# Autodesk Inventor assembly: CaseAssembly
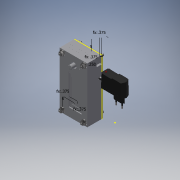
[picture p0: Inventor's stored thumbnail of the model, 180x180]
Saved by Autodesk Inventor 2018 (Build 220112000, 112)
## iProperties
Created: 2020-03-31
Part Number: CaseAssembly
Document SubType Name: Assembly
Designer: emile
Author: emile
## Documents named in this file (11)
- C:\Users\emile\OneDrive\Documents\GitHub\VentilatorCovid19\Respirator\MultiLine\ArduinoCase\CaseAssembly.iam
- C:\Users\emile\OneDrive\Documents\Inventor\Respirator\MultiLine\AC 12V 1A ADAPTER.ipt
- C:\Users\emile\OneDrive\Documents\Inventor\Respirator\MultiLine\ArduinoMega_STEP_AP203.ipt
- C:\Users\emile\OneDrive\Documents\Inventor\Respirator\MultiLine\Ramps 1.4 2004 LCD PRUSA RepRap.ipt
- C:\Users\emile\OneDrive\Documents\Inventor\Respirator\MultiLine\RelayBoard.ipt
- C:\Users\emile\OneDrive\Documents\GitHub\VentilatorCovid19\Respirator\MultiLine\ArduinoCase\FrontPanel.ipt
- C:\Users\emile\OneDrive\Documents\GitHub\VentilatorCovid19\Respirator\MultiLine\ArduinoCase\CaseAssembly\Design Accelerator\Bolted Connection1.iam
- C:\Users\emile\OneDrive\Documents\GitHub\VentilatorCovid19\Respirator\MultiLine\ArduinoCase\RampPanell.ipt
- C:\Users\emile\OneDrive\Documents\GitHub\VentilatorCovid19\Respirator\MultiLine\ArduinoCase\ArduinPanel.ipt
- C:\Users\emile\OneDrive\Documents\GitHub\VentilatorCovid19\Respirator\MultiLine\ArduinoCase\BackCover.ipt
- C:\Users\emile\OneDrive\Documents\GitHub\VentilatorCovid19\Respirator\MultiLine\ArduinoCase\CaseAssembly\Design Accelerator\Bolted Connection3.iam
## Components (10 placed, 9 different names)
1. AC 12V 1A ADAPTER:1 — Mate:14, Mate:15, Angle:1
2. ArduinoMega_STEP_AP203:1 — Flush:6, Mate:12, Mate:14, Mate:15
3. Ramps 1.4 2004 LCD PRUSA RepRap:1 — Mate:2, Mate:3, Mate:5, Flush:1, Mate:6, Mate:10, Flush:4, Flush:5
4. RelayBoard:1 — Mate:16, Flush:7, Mate:17
5. FrontPanel:1 — Mate:2, Mate:3, Mate:4, Flush:1, Mate:8, Flush:2, Flush:3, Mate:9
6. Bolted Connection:1 [sub-assembly] — Mate:4, Mate:5
7. RampPanell:1 — Mate:6, Mate:9, Mate:10, Mate:11
8. ArduinPanel:1 — Flush:4, Mate:11, Flush:5, Flush:6, Mate:12, Mate:16, Flush:7, Mate:17, Angle:1, Mate:18
9. BackCover:1 — Mate:18, Mate:19, Flush:8, Mate:20, Mate:21
10. Bolted Connection:2 [sub-assembly] — Mate:20, Mate:21
## Relationships (27: Mate 18, Flush 8, Angle 1)
- Mate:2: Ramps 1.4 2004 LCD PRUSA RepRap:1 ↔ FrontPanel:1
- Mate:3: Ramps 1.4 2004 LCD PRUSA RepRap:1 ↔ FrontPanel:1
- Mate:4: FrontPanel:1 ↔ Bolted Connection:1
- Mate:5: Ramps 1.4 2004 LCD PRUSA RepRap:1 ↔ Bolted Connection:1
- Flush:1 (1.5875 mm): Ramps 1.4 2004 LCD PRUSA RepRap:1 ↔ FrontPanel:1
- Mate:6: Ramps 1.4 2004 LCD PRUSA RepRap:1 ↔ RampPanell:1
- Mate:8: FrontPanel:1
- Flush:2: FrontPanel:1
- Flush:3: FrontPanel:1
- Mate:9: FrontPanel:1 ↔ RampPanell:1
- Mate:10: Ramps 1.4 2004 LCD PRUSA RepRap:1 ↔ RampPanell:1
- Flush:4: Ramps 1.4 2004 LCD PRUSA RepRap:1 ↔ ArduinPanel:1
- Mate:11: RampPanell:1 ↔ ArduinPanel:1
- Flush:5: Ramps 1.4 2004 LCD PRUSA RepRap:1 ↔ ArduinPanel:1
- Flush:6: ArduinoMega_STEP_AP203:1 ↔ ArduinPanel:1
- Mate:12: ArduinoMega_STEP_AP203:1 ↔ ArduinPanel:1
- Mate:14: AC 12V 1A ADAPTER:1 ↔ ArduinoMega_STEP_AP203:1
- Mate:15: AC 12V 1A ADAPTER:1 ↔ ArduinoMega_STEP_AP203:1
- Mate:16: RelayBoard:1 ↔ ArduinPanel:1
- Flush:7: RelayBoard:1 ↔ ArduinPanel:1
- Mate:17: RelayBoard:1 ↔ ArduinPanel:1
- Angle:1 (180 deg): AC 12V 1A ADAPTER:1 ↔ ArduinPanel:1
- Mate:18: ArduinPanel:1 ↔ BackCover:1
- Mate:19: BackCover:1
- Flush:8: BackCover:1
- Mate:20: BackCover:1 ↔ Bolted Connection:2
- Mate:21: BackCover:1 ↔ Bolted Connection:2
